# Autodesk Inventor assembly: fc17-052
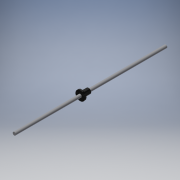
[picture p0: Inventor's stored thumbnail of the model, 180x180]
Saved by Autodesk Inventor 2017.1 (Build 211199000, 199)
## iProperties
Category: Miscellaneous
Company: Autodesk Inc.
Created: 2016-12-16
Part Number: fc17-052
Document SubType Name: Assembly
Designer: Autodesk Inc.
Catalog Web Link: http://www.haydonkerk.com/LinearActuatorProducts/LeadScrewsAndNuts/LeadScrews/tabid/108/Default.aspx
Vendor: Haydon Kerk Motion Solutions
Author: Autodesk Inc.
Keywords: FIRSTChoice
## Documents named in this file (3)
- D:\FIRST\FIRST KOP 2017\FIRST FirstChoice 2017\fc17-052_LeadScrew.iam
- D:\FIRST\FIRST KOP 2017\FIRST FirstChoice 2017\Parts\Ametek-BFWFNR-037-1000-18_1.ipt
- D:\FIRST\FIRST KOP 2017\FIRST FirstChoice 2017\Parts\Ametek-BFWFNR-037-1000-18_2.ipt
## Components (2 placed, 2 different names)
1. Ametek-BFWFNR-037-1000-18_1:1 — Mate:1
2. Ametek-BFWFNR-037-1000-18_2:1 — Mate:1
## Relationships (1: Mate 1)
- Mate:1: Ametek-BFWFNR-037-1000-18_1:1 ↔ Ametek-BFWFNR-037-1000-18_2:1
